# Autodesk Inventor assembly: presentation flip
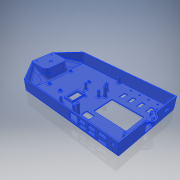
[picture p0: Inventor's stored thumbnail of the model, 180x180]
Saved by Autodesk Inventor 2019 (Build 230136000, 136)
## iProperties
Created: 2020-02-21
Part Number: presentation flip
Document SubType Name: Assembly
Designer: close
Author: close
## Documents named in this file (2)
- C:\Users\close\Desktop\CAD BARC-ROAR\barc_hardware\Enclosure\V_3\presentation flip.iam
- C:\Users\close\Desktop\CAD BARC-ROAR\barc_hardware\Enclosure\V_3\Enclosure_v3.ipt
## Components (1 placed, 1 different names)
1. Enclosure_v3:1 — Mate:1
## Relationships (1: Mate 1)
- Mate:1: Enclosure_v3:1
